# Autodesk Inventor assembly: Lab3_Ex1_temp
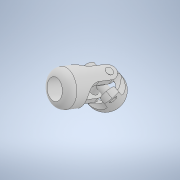
[picture p0: Inventor's stored thumbnail of the model, 180x180]
Saved by Autodesk Inventor 2022 (Build 260153000, 153)
## iProperties
Created: 2022-01-27
Part Number: Lab3_Ex1_temp
Document SubType Name: Assembly
Designer: Administrator
Title: Lab3_Ex1_temp v4
Author: Administrator
## Documents named in this file (3)
- C:\Users\br4ch\M-and-Ms\HW2\Task1\Inventor\Lab3_Ex1_temp.iam
- C:\Users\br4ch\M-and-Ms\HW2\Task1\Inventor\element_a.ipt
- C:\Users\br4ch\M-and-Ms\HW2\Task1\Inventor\element_a (1).ipt
## Components (3 placed, 2 different names)
1. element_a:1 — Mate:1, Rotational:1
2. element_a (1):1 — Mate:1, Rotational:1, Rotational:2
3. element_a:2 — Rotational:2
## Relationships (3: RevoluteJoint 2, Mate 1)
- Mate:1: element_a:1 ↔ element_a (1):1
- Rotational:1 [RevoluteJoint]: element_a:1 ↔ element_a (1):1
- Rotational:2 [RevoluteJoint]: element_a (1):1 ↔ element_a:2
